# Autodesk Inventor assembly: Race Inner
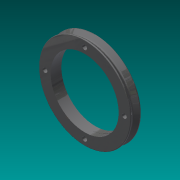
[picture p0: Inventor's stored thumbnail of the model, 180x180]
Saved by Autodesk Inventor 2020.3 (Build 243373000, 373)
## iProperties
Created: 2020-05-24
Part Number: Race Inner
Document SubType Name: Assembly
Designer: Administrator
Title: Race Inner
Author: Administrator
## Documents named in this file (3)
- C:\Users\Svend\OneDrive\Documents\GitHub\BeerMinder\3D-model\bearings\slew bearing 80 mm\Race Inner - 80mm.iam
- C:\Users\Svend\OneDrive\Documents\GitHub\BeerMinder\3D-model\bearings\slew bearing 80 mm\Race Inner Bottom - 80mm.ipt
- C:\Users\Svend\OneDrive\Documents\GitHub\BeerMinder\3D-model\bearings\slew bearing 80 mm\Race Inner Top - 80mm.ipt
## Components (2 placed, 2 different names)
1. Race Inner Bottom - 80mm:1 — Mate:1, Mate:2, Mate:3
2. Race Inner Top - 80mm:1 — Mate:1, Mate:2, Mate:3
## Relationships (3: Mate 3)
- Mate:1: Race Inner Bottom - 80mm:1 ↔ Race Inner Top - 80mm:1
- Mate:2: Race Inner Bottom - 80mm:1 ↔ Race Inner Top - 80mm:1
- Mate:3: Race Inner Bottom - 80mm:1 ↔ Race Inner Top - 80mm:1
